# Autodesk Inventor assembly: BottomPart
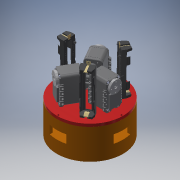
[picture p0: Inventor's stored thumbnail of the model, 180x180]
Saved by Autodesk Inventor 2019 (Build 230136000, 136)
## iProperties
Created: 2022-07-05
Part Number: BottomPart
Document SubType Name: Assembly
Designer: zreik
Author: zreik
## Documents named in this file (5)
- D:\Documents\HIAST\4th year\4th Year Project\Design\BottomPart.iam
- D:\Documents\HIAST\4th year\4th Year Project\Design\Base.ipt
- D:\Documents\HIAST\4th year\4th Year Project\Design\Cover.ipt
- D:\Documents\HIAST\4th year\4th Year Project\Design\AX-12A\AX-12A.iam
- D:\Documents\HIAST\4th year\4th Year Project\Design\BatteryHolder.ipt
## Components (8 placed, 4 different names)
1. Base:1 — Mate:1, Mate:2, Mate:3
2. Cover:1 — Mate:1, Mate:2, Mate:3, Mate:4, Mate:5, Mate:6, Mate:7, Mate:9, Mate:10
3. AX-12A:1 [sub-assembly] — Mate:6, Angle:1
4. AX-12A:2 [sub-assembly] — Mate:5, Angle:1, Angle:2, Angle:5
5. AX-12A:3 [sub-assembly] — Mate:4, Angle:2
6. BatteryHolder:1 — Angle:3, Mate:9, Angle:5
7. BatteryHolder:2 — Angle:3, Angle:4, Mate:10
8. BatteryHolder:3 — Angle:4, Mate:7
## Relationships (14: Mate 9, Angle 5)
- Mate:1: Base:1 ↔ Cover:1
- Mate:2: Base:1 ↔ Cover:1
- Mate:3: Base:1 ↔ Cover:1
- Mate:4: Cover:1 ↔ AX-12A:3
- Mate:5: Cover:1 ↔ AX-12A:2
- Mate:6: Cover:1 ↔ AX-12A:1
- Angle:1 (120 deg): AX-12A:1 ↔ AX-12A:2
- Angle:2 (120 deg): AX-12A:2 ↔ AX-12A:3
- Angle:3 (120 deg): BatteryHolder:1 ↔ BatteryHolder:2
- Angle:4 (-120 deg): BatteryHolder:2 ↔ BatteryHolder:3
- Mate:7: Cover:1 ↔ BatteryHolder:3
- Mate:9: Cover:1 ↔ BatteryHolder:1
- Mate:10: Cover:1 ↔ BatteryHolder:2
- Angle:5 (60 deg): AX-12A:2 ↔ BatteryHolder:1
